# Autodesk Inventor assembly: mount
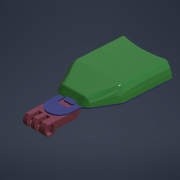
[picture p0: Inventor's stored thumbnail of the model, 180x180]
Saved by Autodesk Inventor 2022 (Build 260153000, 153)
## iProperties
Part Number: mount
Document SubType Name: Assembly
Designer: ancher
Author: ancher
## Documents named in this file (4)
- E:\RC\print_3d\cobrax_mount\mount.iam
- E:\RC\print_3d\cobrax_mount\latch.ipt
- E:\RC\print_3d\cobrax_mount\cap.ipt
- E:\RC\print_3d\cobrax_mount\gopro.ipt
## Components (3 placed, 3 different names)
1. latch:1 — Flush:1, Rigid:1
2. cap:1 — Flush:1
3. gopro:1 — Rigid:1
## Relationships (2: Flush 1, WeldJoint 1)
- Flush:1: latch:1 ↔ cap:1
- Rigid:1 [WeldJoint]: latch:1 ↔ gopro:1
